# Autodesk Inventor assembly: 000.003 - Блок АКБ СБ
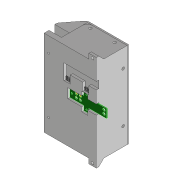
[picture p0: Inventor's stored thumbnail of the model, 180x180]
Saved by Autodesk Inventor 2022 (Build 260153000, 153)
## iProperties
Created: 2022-02-26
Part Number: 000.003 - Блок АКБ СБ
Document SubType Name: Assembly
Designer: Petrov Ivan
Mass: 725.732 g
Surface Area: 2626.29 cm^2
Volume: 725.732 cm^3
Density: 1 g/cm^3
Author: Petrov Ivan
## Documents named in this file (7)
- C:\Users\Ivan Petrov\Documents\GitHub\OmniBot\design\000.003 - Блок АКБ СБ.iam
- C:\Users\Ivan Petrov\Documents\GitHub\OmniBot\design\000.003.001 - Основание.ipt
- C:\Users\Ivan Petrov\Documents\GitHub\OmniBot\design\standart_components\NUCLEO.ipt
- C:\Users\Ivan Petrov\Documents\GitHub\OmniBot\design\standart_components\connectrs\JST - XH - Thru (R) - 4Pin - 2.54mm.ipt
- C:\Users\Ivan Petrov\Documents\GitHub\OmniBot\design\standart_components\XT60FemaleConnector.ipt
- C:\Users\Ivan Petrov\Documents\GitHub\OmniBot\electronic\xt60_pcb\3d_model\xt60_pcb.brdКонтур.ipt
- C:\Users\Ivan Petrov\Documents\GitHub\OmniBot\design\Docs\000.003.002 - Крышка.ipt
## Components (9 placed, 6 different names)
1. 000.003.001 - Основание.ipt:1 — Совмещение:2, Совмещение:3, Заподлицо:2, Совмещение:4, Совмещение:5, Заподлицо:3, Совмещение:6, Совмещение:7, Касательность:1, Касательность:2, Совмещение:8, Совмещение:9, Совмещение:11, Угол:1, Совмещение:13, Совмещение:14, Заподлицо:7, Заподлицо:8
2. NUCLEO.ipt:1 — Совмещение:6, Касательность:2, Заподлицо:4
3. NUCLEO.ipt:2 — Совмещение:7, Касательность:1, Заподлицо:4
4. JST - XH - Thru (R) - 4Pin - 2.54mm:1 — Совмещение:4, Совмещение:5, Заподлицо:3
5. JST - XH - Thru (R) - 4Pin - 2.54mm:2 — Совмещение:2, Совмещение:3, Заподлицо:2
6. XT60FemaleConnector:1 — Совмещение:8, Совмещение:9, Совмещение:10, Заподлицо:6, Совмещение:12
7. XT60FemaleConnector:2 — Совмещение:10, Совмещение:11, Заподлицо:6
8. xt60_pcb.brdКонтур:1 — Совмещение:12, Угол:1, Совмещение:13
9. 000.003.002 - Крышка:1 — Совмещение:14, Заподлицо:7, Заподлицо:8
## Relationships (22: Mate 13, Flush 6, Tangent 2, Angle 1)
- Совмещение:2 [Mate]: 000.003.001 - Основание.ipt:1 ↔ JST - XH - Thru (R) - 4Pin - 2.54mm:2
- Совмещение:3 [Mate]: 000.003.001 - Основание.ipt:1 ↔ JST - XH - Thru (R) - 4Pin - 2.54mm:2
- Заподлицо:2 [Flush]: 000.003.001 - Основание.ipt:1 ↔ JST - XH - Thru (R) - 4Pin - 2.54mm:2
- Совмещение:4 [Mate]: 000.003.001 - Основание.ipt:1 ↔ JST - XH - Thru (R) - 4Pin - 2.54mm:1
- Совмещение:5 [Mate]: 000.003.001 - Основание.ipt:1 ↔ JST - XH - Thru (R) - 4Pin - 2.54mm:1
- Заподлицо:3 [Flush]: 000.003.001 - Основание.ipt:1 ↔ JST - XH - Thru (R) - 4Pin - 2.54mm:1
- Совмещение:6 [Mate] (5 mm): 000.003.001 - Основание.ipt:1 ↔ NUCLEO.ipt:1
- Совмещение:7 [Mate] (5 mm): 000.003.001 - Основание.ipt:1 ↔ NUCLEO.ipt:2
- Касательность:1 [Tangent]: 000.003.001 - Основание.ipt:1 ↔ NUCLEO.ipt:2
- Касательность:2 [Tangent]: 000.003.001 - Основание.ipt:1 ↔ NUCLEO.ipt:1
- Заподлицо:4 [Flush]: NUCLEO.ipt:1 ↔ NUCLEO.ipt:2
- Совмещение:8 [Mate]: 000.003.001 - Основание.ipt:1 ↔ XT60FemaleConnector:1
- Совмещение:9 [Mate]: 000.003.001 - Основание.ipt:1 ↔ XT60FemaleConnector:1
- Совмещение:10 [Mate]: XT60FemaleConnector:1 ↔ XT60FemaleConnector:2
- Совмещение:11 [Mate]: 000.003.001 - Основание.ipt:1 ↔ XT60FemaleConnector:2
- Заподлицо:6 [Flush]: XT60FemaleConnector:1 ↔ XT60FemaleConnector:2
- Совмещение:12 [Mate]: XT60FemaleConnector:1 ↔ xt60_pcb.brdКонтур:1
- Угол:1 [Angle] (0 deg): 000.003.001 - Основание.ipt:1 ↔ xt60_pcb.brdКонтур:1
- Совмещение:13 [Mate]: 000.003.001 - Основание.ipt:1 ↔ xt60_pcb.brdКонтур:1
- Совмещение:14 [Mate]: 000.003.001 - Основание.ipt:1 ↔ 000.003.002 - Крышка:1
- Заподлицо:7 [Flush]: 000.003.001 - Основание.ipt:1 ↔ 000.003.002 - Крышка:1
- Заподлицо:8 [Flush]: 000.003.001 - Основание.ipt:1 ↔ 000.003.002 - Крышка:1
